# Autodesk Inventor assembly: Container
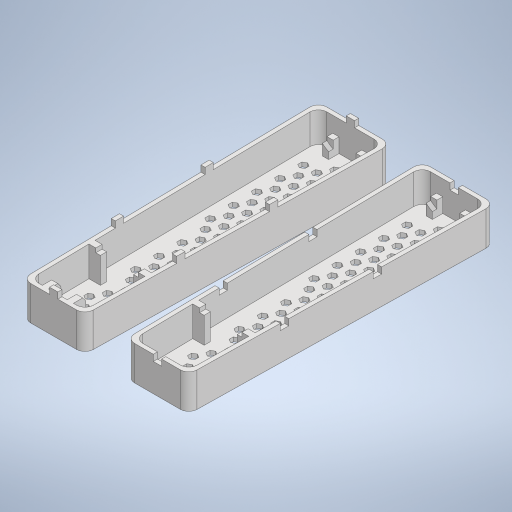
[picture p0: Inventor's stored thumbnail of the model, 512x512]
Saved by Autodesk Inventor 2023 (Build 270158000, 158)
## iProperties
Created: 2022-11-17
Part Number: Container
Document SubType Name: Assembly
Designer: The-M-Factor
Author: The-M-Factor
## Documents named in this file (3)
- G:\Other computers\MattLaptop\FirstYearLectures\1P13\DesignStudios\P2\Milestone 4\Container.iam
- G:\Other computers\MattLaptop\FirstYearLectures\1P13\DesignStudios\P2\Milestone 3\ContainerBottom.ipt
- G:\Other computers\MattLaptop\FirstYearLectures\1P13\DesignStudios\P2\Milestone 3\ContainerTop.ipt
## Components (2 placed, 2 different names)
1. ContainerBottom:1 — Flush:1, Flush:2, Flush:3
2. ContainerTop:1 — Flush:1, Flush:2, Flush:3
## Relationships (3: Flush 3)
- Flush:1: ContainerBottom:1 ↔ ContainerTop:1
- Flush:2: ContainerBottom:1 ↔ ContainerTop:1
- Flush:3 (50 mm): ContainerBottom:1 ↔ ContainerTop:1
